# Autodesk Inventor assembly: Fanduct
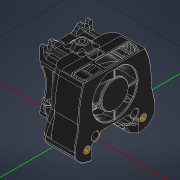
[picture p0: Inventor's stored thumbnail of the model, 180x180]
Saved by Autodesk Inventor 2022.2 (Build 262287010, 287A)
## iProperties
Created: 2022-03-16
Part Number: Fanduct
Document SubType Name: Assembly
Designer: sleib
Author: sleib
## Documents named in this file (5)
- C:\Users\sleib\Projekte\Voron-2\CAD\Inventor\Afterburner\Fanduct-Unit.iam
- C:\Users\sleib\Projekte\Voron-2\CAD\Inventor\Afterburner\Hotend Back.ipt
- C:\Users\sleib\Projekte\Voron-2\CAD\Inventor\Afterburner\Hotend Fanduct.ipt
- C:\Users\sleib\Projekte\Voron-2\CAD\Inventor\M3 Threaded Insert.ipt
- C:\Users\sleib\Projekte\Voron-2\CAD\Inventor\Dragon Hotend\Dragon Hotend.iam
## Components (5 placed, 4 different names)
1. Hotend Back:1 — Fluchtend:1, Passend:1, Passend:2, Passend:3, Fluchtend:2
2. Hotend Fanduct:1 — Fluchtend:1, Passend:1, Passend:2, Passend:3, Fluchtend:2, Passend:4, Passend:5, Fluchtend:3, Fluchtend:4, Passend:6, Passend:7, Passend:8
3. M3 Threaded Insert:1 — Passend:4, Fluchtend:4
4. M3 Threaded Insert:2 — Passend:5, Fluchtend:3
5. Dragon Hotend:1 [sub-assembly] — Passend:6, Passend:7, Passend:8
## Relationships (12: Mate 8, Flush 4)
- Fluchtend:1 [Flush]: Hotend Back:1 ↔ Hotend Fanduct:1
- Passend:1 [Mate]: Hotend Back:1 ↔ Hotend Fanduct:1
- Passend:2 [Mate]: Hotend Back:1 ↔ Hotend Fanduct:1
- Passend:3 [Mate]: Hotend Back:1 ↔ Hotend Fanduct:1
- Fluchtend:2 [Flush]: Hotend Back:1 ↔ Hotend Fanduct:1
- Passend:4 [Mate]: Hotend Fanduct:1 ↔ M3 Threaded Insert:1
- Passend:5 [Mate]: Hotend Fanduct:1 ↔ M3 Threaded Insert:2
- Fluchtend:3 [Flush]: Hotend Fanduct:1 ↔ M3 Threaded Insert:2
- Fluchtend:4 [Flush]: Hotend Fanduct:1 ↔ M3 Threaded Insert:1
- Passend:6 [Mate]: Hotend Fanduct:1 ↔ Dragon Hotend:1
- Passend:7 [Mate]: Hotend Fanduct:1 ↔ Dragon Hotend:1
- Passend:8 [Mate]: Hotend Fanduct:1 ↔ Dragon Hotend:1
